# Autodesk Inventor assembly: master_assembly_1
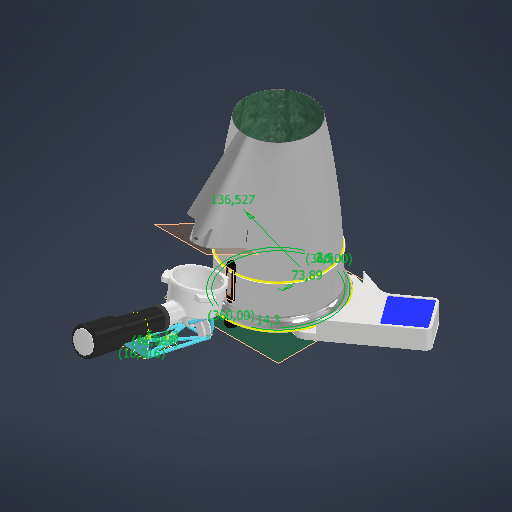
[picture p0: Inventor's stored thumbnail of the model, 512x512]
Saved by Autodesk Inventor 2026 (Build 300175000, 175)
## iProperties
Created: 2025-05-05
Part Number: master_assembly_1
Document SubType Name: Assembly
Designer: Paul Juschitz
Author: Paul Juschitz
## Documents named in this file (11)
- C:\Users\Paul Juschitz\Documents\private\m5_GBW_mod\M5_GBW_mod\CAD\master\master_assembly_1.iam
- C:\Users\Paul Juschitz\Documents\private\m5_GBW_mod\M5_GBW_mod\CAD\master\m2m_shell_3.ipt
- C:\Users\Paul Juschitz\Documents\private\m5_GBW_mod\M5_GBW_mod\CAD\master\m2m_bottom_2.ipt
- C:\Users\Paul Juschitz\Documents\private\m5_GBW_mod\M5_GBW_mod\CAD\master\my_portafilter_holder_8.ipt
- C:\Users\Paul Juschitz\Documents\private\m5_GBW_mod\M5_GBW_mod\CAD\master\load_cell.ipt
- C:\Users\Paul Juschitz\Documents\private\m5_GBW_mod\M5_GBW_mod\CAD\master\BES870XL Portafilter\BES870XL Portafilter_assembled.iam
- C:\Users\Paul Juschitz\Documents\private\m5_GBW_mod\M5_GBW_mod\CAD\master\mock_dosing_funnel.ipt
- C:\Users\Paul Juschitz\Documents\private\m5_GBW_mod\M5_GBW_mod\CAD\master\load_cell_holder_1.ipt
- C:\Users\Paul Juschitz\Documents\private\m5_GBW_mod\M5_GBW_mod\CAD\master\core_dummy_1.ipt
- C:\Users\Paul Juschitz\Documents\private\m5_GBW_mod\M5_GBW_mod\CAD\master\core_housing_bottom_1.ipt
- C:\Users\Paul Juschitz\Documents\private\m5_GBW_mod\M5_GBW_mod\CAD\master\core_housing_top_1.ipt
## Components (10 placed, 10 different names)
1. m2m_shell_3:1 — Mate:1, Mate:2, Mate:3, Mate:7, Tangent:3
2. m2m_bottom_2:1 — Mate:2, Mate:3, Flush:6, Cylindrical:1, Cylindrical:2, Mate:23
3. my_portafilter_holder_8:1 — Flush:5, Angle:1, Tangent:1, Tangent:2, Mate:16, Mate:17
4. load_cell:1 — Mate:16, Mate:17, Mate:18
5. BES870XL Portafilter_assembled:1 [sub-assembly] — Mate:4, Angle:1, Tangent:1, Tangent:2, Mate:6
6. mock_dosing_funnel:1 — Mate:6
7. load_cell_holder_1:1 — Mate:7, Tangent:3, Mate:18
8. core_housing_bottom_1:1 — Mate:19, Mate:20, Mate:21, Mate:22
9. core_housing_top_1:1 — Mate:21, Mate:22, Cylindrical:1, Cylindrical:2, Mate:23
10. core_dummy_1:1 — Mate:19, Mate:20
## Relationships (22: Mate 14, Tangent 3, Flush 2, CylindricalJoint 2, Angle 1)
- Mate:1: m2m_shell_3:1
- Mate:2: m2m_shell_3:1 ↔ m2m_bottom_2:1
- Mate:3: m2m_shell_3:1 ↔ m2m_bottom_2:1
- Flush:5: my_portafilter_holder_8:1
- Mate:4: BES870XL Portafilter_assembled:1
- Angle:1 (180 deg): my_portafilter_holder_8:1 ↔ BES870XL Portafilter_assembled:1
- Tangent:1: my_portafilter_holder_8:1 ↔ BES870XL Portafilter_assembled:1
- Tangent:2: my_portafilter_holder_8:1 ↔ BES870XL Portafilter_assembled:1
- Mate:6: BES870XL Portafilter_assembled:1 ↔ mock_dosing_funnel:1
- Mate:7: m2m_shell_3:1 ↔ load_cell_holder_1:1
- Tangent:3: m2m_shell_3:1 ↔ load_cell_holder_1:1
- Mate:16: my_portafilter_holder_8:1 ↔ load_cell:1
- Mate:17: my_portafilter_holder_8:1 ↔ load_cell:1
- Mate:18: load_cell:1 ↔ load_cell_holder_1:1
- Flush:6: m2m_bottom_2:1
- Mate:19: core_housing_bottom_1:1 ↔ core_dummy_1:1
- Mate:20: core_housing_bottom_1:1 ↔ core_dummy_1:1
- Mate:21: core_housing_bottom_1:1 ↔ core_housing_top_1:1
- Mate:22: core_housing_bottom_1:1 ↔ core_housing_top_1:1
- Cylindrical:1: m2m_bottom_2:1 ↔ core_housing_top_1:1
- Cylindrical:2: m2m_bottom_2:1 ↔ core_housing_top_1:1
- Mate:23: m2m_bottom_2:1 ↔ core_housing_top_1:1
## Named parameters: m2m_bottom_radius_lower = 76 mm, m2m_bottom_radius_upper = 68 mm, m2m_top_radius = 48 mm, m2m_shell_thickness = 0.5 mm, m2m_shell_height = 220 mm, m2m_shell_base_height = 16 mm, m2m_shell_bottom_screwhole_inset = -2 mm, m2m_shell_bottom_screwhole_ID = 2.5 mm, m2m_shell_bottom_screwhole_OD = 3.9 mm, m2m_spout_height_inner = 93 mm, m2m_spout_height_outer = 121 mm, m2m_spout_angle = 27.5 deg, m2m_opening_bracket_outer_width = 20 mm, m2m_center_radius = 136.52735 mm, m2m_fork_bracket_outer_thickness = 3.8 mm, m2m_fork_bracket_inner_thickness = 0 mm, m2m_fork_bracket_height_bottom = 20.6 mm, m2m_fork_bracket_height = 50.4 mm, m2m_shell_spout_diameter = 30.6 mm
